# Autodesk Inventor assembly: tire form
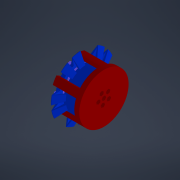
[picture p0: Inventor's stored thumbnail of the model, 180x180]
Saved by Autodesk Inventor 2022 (Build 260153000, 153)
## iProperties
Created: 2023-02-07
Part Number: tire form
Document SubType Name: Assembly
Designer: akapu
Author: akapu
## Documents named in this file (5)
- C:\Users\akapu\OneDrive\Документы\maze bot\tire form.iam
- C:\Users\akapu\OneDrive\Документы\maze bot\tire.ipt
- C:\Users\akapu\OneDrive\Документы\maze bot\tire ring.ipt
- C:\Users\akapu\OneDrive\Документы\maze bot\tire disk.ipt
- C:\Users\akapu\OneDrive\Документы\maze bot\tire cap.ipt
## Components (4 placed, 4 different names)
1. tire:1 — Совмещение:1, С поворотом:1, Заподлицо:3
2. tire ring:1 — Совмещение:1, С поворотом:1, Заподлицо:1
3. tire disk:1 — Заподлицо:1, Заподлицо:2
4. tire cap:1 — Заподлицо:2
## Relationships (5: Flush 3, Mate 1, RevoluteJoint 1)
- Совмещение:1 [Mate]: tire:1 ↔ tire ring:1
- С поворотом:1 [RevoluteJoint]: tire:1 ↔ tire ring:1
- Заподлицо:1 [Flush]: tire ring:1 ↔ tire disk:1
- Заподлицо:2 [Flush]: tire disk:1 ↔ tire cap:1
- Заподлицо:3 [Flush]: tire:1
